# Autodesk Inventor assembly: ASY GBK 1310 long wall shield 4
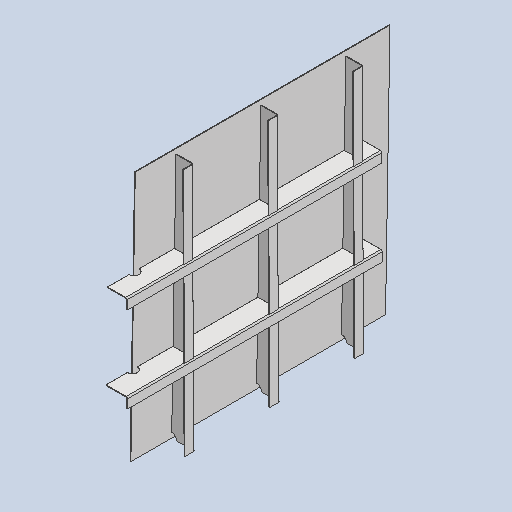
[picture p0: Inventor's stored thumbnail of the model, 512x512]
Saved by Autodesk Inventor 2026.2 (Build 302298000, 298)
## iProperties
Created: 2026-05-07
Part Number: ASY GBK 1310 long wall shield 4
Document SubType Name: Assembly
Designer: pokla
Mass: 107756 g
Surface Area: 69611.7 cm^2
Volume: 13726.9 cm^3
Density: 7.85 g/cm^3
Author: admin
## Documents named in this file (6)
- C:\Users\admin\Documents\Inventor\GBK-Gubkinskiy\ASY GBK 1310 long wall shield 4.iam
- C:\Users\admin\Documents\Inventor\GBK-Gubkinskiy\07.1 GBK shield.ipt
- C:\Users\admin\Documents\Inventor\GBK-Gubkinskiy\07.2 GBK rib.ipt
- C:\Users\admin\Documents\Inventor\GBK-Gubkinskiy\0371 GBK stringer 7.ipt
- C:\Users\admin\Documents\Inventor\GBK-Gubkinskiy\0372 GBK stringer 8.ipt
- C:\Users\admin\Documents\Inventor\GBK-Gubkinskiy\GBK 1111 main rib.ipt
## Components (6 placed, 4 different names)
1. GBK 1312 stringer 7:1
2. GBK 1313 stringer 8:1
3. CH 1019 GBK shield:1
4. GBK 1311 third rib:1
5. GBK 1311 third rib:2
6. GBK 1311 third rib:3
## Component patterns: (3 elements, first: GBK 1311 third rib:1)
## Relationships (5: Mate 2, WeldJoint 2, Flush 1)
- [Flush] (254 mm): CH 1019 GBK shield:1 ↔ GBK 1311 third rib:1
- [Mate]: CH 1019 GBK shield:1 ↔ GBK 1311 third rib:1
- [Mate]: CH 1019 GBK shield:1 ↔ GBK 1311 third rib:1
- [WeldJoint] (4 mm): GBK 1312 stringer 7:1 ↔ GBK 1311 third rib:1
- [WeldJoint] (4 mm): GBK 1313 stringer 8:1 ↔ GBK 1311 third rib:1
## Named parameters: Шаг_шпангоутов = 496.66667 mm
